# Autodesk Inventor assembly: vitme_aogoi
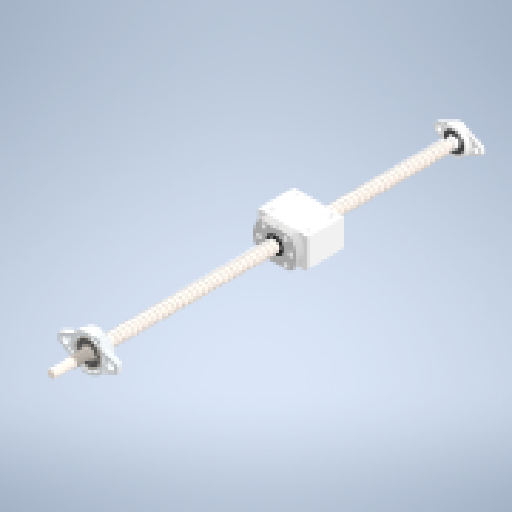
[picture p0: Inventor's stored thumbnail of the model, 512x512]
Saved by Autodesk Inventor 2023 (Build 270158000, 158)
## iProperties
Created: 2025-04-10
Part Number: vitme_aogoi
Document SubType Name: Assembly
Designer: LENOVO
Author: LENOVO
## Documents named in this file (6)
- E:\TAI LIEU\Final_Project\DONE\CoCauTrucZ\vitme_aogoi\vitme_aogoi.iam
- E:\TAI LIEU\Final_Project\DONE\CoCauTrucZ\vitme_aogoi\Generic Ballscrew\Generic Ballscrew.ipt
- E:\TAI LIEU\Final_Project\DONE\CoCauTrucZ\vitme_aogoi\SFU1204 Nut v1\SFU1204 Nut v1.ipt
- E:\TAI LIEU\Final_Project\DONE\CoCauTrucZ\vitme_aogoi\dsg 12 v2\dsg 12 v2.ipt
- E:\TAI LIEU\Final_Project\DONE\CoCauTrucZ\vitme_aogoi\KFL000 bearing unit 10mm\KFL000 bearing unit 10mm.ipt
- E:\TAI LIEU\Final_Project\DONE\CoCauTrucZ\vitme_aogoi\KFL08 - Mancal Flange oval Ø8\KFL08 - Mancal Flange oval Ø8.ipt
## Components (5 placed, 5 different names)
1. Generic Ballscrew:1 — Mate:1, Mate:5, Mate:7, Flush:1
2. SFU1204 Nut v1:1 — Mate:1, Mate:2, Mate:3, Mate:4
3. dsg 12 v2:1 — Mate:2, Mate:3, Mate:4, Flush:2
4. KFL000 bearing unit 10mm:1 — Mate:5, Mate:8, Flush:1
5. KFL08 - Mancal Flange oval Ø8:1 — Mate:7, Mate:8, Flush:2
## Relationships (9: Mate 7, Flush 2)
- Mate:1: Generic Ballscrew:1 ↔ SFU1204 Nut v1:1
- Mate:2: SFU1204 Nut v1:1 ↔ dsg 12 v2:1
- Mate:3: SFU1204 Nut v1:1 ↔ dsg 12 v2:1
- Mate:4: SFU1204 Nut v1:1 ↔ dsg 12 v2:1
- Mate:5: Generic Ballscrew:1 ↔ KFL000 bearing unit 10mm:1
- Mate:7: Generic Ballscrew:1 ↔ KFL08 - Mancal Flange oval Ø8:1
- Mate:8 (-370 mm): KFL000 bearing unit 10mm:1 ↔ KFL08 - Mancal Flange oval Ø8:1
- Flush:1 (16 mm): Generic Ballscrew:1 ↔ KFL000 bearing unit 10mm:1
- Flush:2 (134.55 mm): dsg 12 v2:1 ↔ KFL08 - Mancal Flange oval Ø8:1
